# Autodesk Inventor assembly: SAD
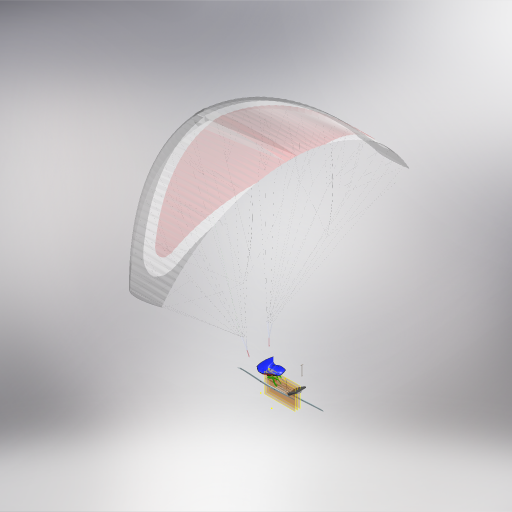
[picture p0: Inventor's stored thumbnail of the model, 512x512]
Saved by Autodesk Inventor 2024 (Build 280153000, 153)
## iProperties
Created: 2023-10-22
Part Number: SAD
Document SubType Name: Assembly
Designer: tinas
Author: tinas
## Documents named in this file (10)
- C:\Users\tinas\OneDrive\Desktop\SpeedRiding\SpeedRiding\CAD\As\SAD.iam
- C:\Users\tinas\OneDrive\Desktop\SpeedRiding\SpeedRiding\CAD\Sit\Sit.ipt
- C:\Users\tinas\OneDrive\Desktop\SpeedRiding\SpeedRiding\CAD\As\SHOCK ASSEMBLY.iam
- C:\Users\tinas\OneDrive\Desktop\SpeedRiding\SpeedRiding\CAD\As\Frame Assembly.iam
- C:\Users\tinas\OneDrive\Desktop\SpeedRiding\SpeedRiding\CAD\As\BASE.ipt
- C:\Users\tinas\OneDrive\Desktop\SpeedRiding\SpeedRiding\CAD\Wing\Wing.iam
- C:\Users\tinas\OneDrive\Desktop\SpeedRiding\SpeedRiding\CAD\As\CONNECTION BAR SHORT_Default_As Machined_.ipt
- C:\Users\tinas\OneDrive\Desktop\SpeedRiding\SpeedRiding\CAD\As\CONNECTION BAR_Default_As Machined_.ipt
- C:\Users\tinas\OneDrive\Desktop\SpeedRiding\SpeedRiding\CAD\FINAL ASSEMBLY v1\FOOT REST.ipt
- C:\Users\tinas\OneDrive\Desktop\SpeedRiding\SpeedRiding\CAD\Skii\SKC\SKC.iam
## Components (11 placed, 9 different names)
1. Sit:1
2. SHOCK ASSEMBLY:2 [sub-assembly]
3. Frame Assembly:1 [sub-assembly]
4. BASE:1 — Rotation:1, Mate:1
5. Wing:1 [sub-assembly]
6. CONNECTION BAR SHORT_Default_As Machined_:1
7. CONNECTION BAR_Default_As Machined_:1 — Rotation:1, Mate:1
8. CONNECTION BAR SHORT_Default_As Machined_:2
9. FOOT REST:1
10. SKC:1 [sub-assembly]
11. SKC:2 [sub-assembly]
## Relationships (2: RelateRotation 1, Mate 1)
- Rotation:1 [RelateRotation] (1 ul): BASE:1 ↔ CONNECTION BAR_Default_As Machined_:1
- Mate:1: BASE:1 ↔ CONNECTION BAR_Default_As Machined_:1
